# Autodesk Inventor assembly: Крепление датчика ульразвука
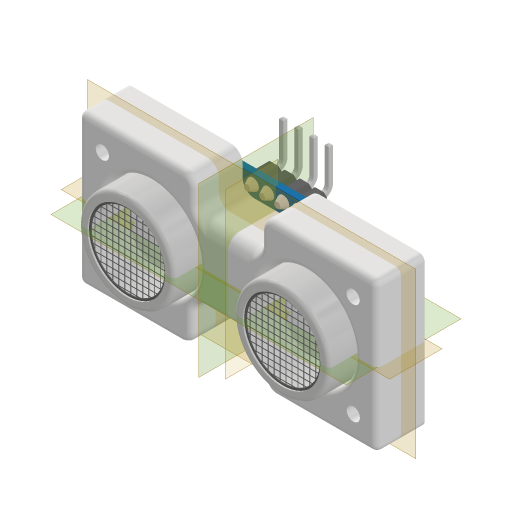
[picture p0: Inventor's stored thumbnail of the model, 512x512]
Saved by Autodesk Inventor 2023.2 (Build 272271030, 271C)
## iProperties
Created: 2025-05-24
Part Number: Крепление датчика ульразвука
Document SubType Name: Assembly
Designer: Олег Коноваленко
Author: Олег Коноваленко
## Documents named in this file (3)
- D:\!Rover\Rover\Rover_construction\Крепление датчика ульразвука.iam
- D:\!Rover\Rover\Rover_construction\HC-04HC-04\HC-04HC-04.iam
- D:\!Rover\Rover\Rover_construction\Крепление_ультразвука.ipt
## Components (2 placed, 2 different names)
1. HC-04HC-04:1 [sub-assembly] — Совмещение:3, Совмещение:4, Совмещение:5, Совмещение:6, Совмещение:7
2. Крепление_ультразвука:1 — Совмещение:5, Совмещение:6, Совмещение:7
## Relationships (5: Mate 5)
- Совмещение:3 [Mate]: HC-04HC-04:1
- Совмещение:4 [Mate]: HC-04HC-04:1
- Совмещение:5 [Mate]: HC-04HC-04:1 ↔ Крепление_ультразвука:1
- Совмещение:6 [Mate]: HC-04HC-04:1 ↔ Крепление_ультразвука:1
- Совмещение:7 [Mate]: HC-04HC-04:1 ↔ Крепление_ультразвука:1
